# Autodesk Inventor assembly: DelrinX-Wheel-Top_MIR
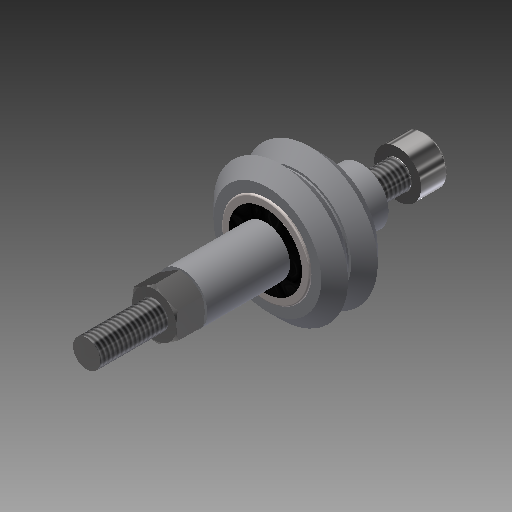
[picture p0: Inventor's stored thumbnail of the model, 512x512]
Saved by Autodesk Inventor 2017 (Build 210142000, 142)
## iProperties
Created: 2016-07-20
Part Number: DelrinX-Wheel-Top_MIR
Document SubType Name: Assembly
Designer: User
Author: User
## Documents named in this file (6)
- C:\All INVENTOR\SL-Inventor\SL-Beast 3D Printer\DelrinX-Wheel-Top_MIR.iam
- C:\All INVENTOR\SL-Inventor\SL-Beast 3D Printer\DelrinWheel_MIR.iam
- C:\All INVENTOR\SL-Inventor\SL-Beast 3D Printer\Long-Spacer_MIR.ipt
- C:\All INVENTOR\SL-Inventor\SL-Beast 3D Printer\ANSI B18.3.1M - M5x0.8 x 60NEW_MIR.ipt
- C:\All INVENTOR\SL-Inventor\SL-Beast 3D Printer\en-US\ANSI B 18.2.4.1 M(1)\ANSI B 18.2.4.1 M - M5 x 0.8Style 2.ipt
- C:\All INVENTOR\SL-Inventor\SL-Beast 3D Printer\Small-Aluminium-Spacer_MIR1.ipt
## Components (5 placed, 5 different names)
1. DelrinWheel_MIR:1 [sub-assembly] — Mate:2, Mate:1, Flush:1
2. Long-Spacer_MIR:1 — Insert:1
3. ANSI B18.3.1M - M5x0.8 x 60NEW_MIR:1 — Mate:2, Mate:1
4. Hex Nut Metric M5 x 0.8:1 — Insert:1
5. Small-Aluminium-Spacer_MIR1:1 — Flush:1
## Relationships (4: Mate 3, Insert 1)
- Mate:2 (13 mm): DelrinWheel_MIR:1 ↔ ANSI B18.3.1M - M5x0.8 x 60NEW_MIR:1
- Mate:1: DelrinWheel_MIR:1 ↔ ANSI B18.3.1M - M5x0.8 x 60NEW_MIR:1
- Insert:1: Long-Spacer_MIR:1 ↔ Hex Nut Metric M5 x 0.8:1
- Flush:1 [Mate]: DelrinWheel_MIR:1 ↔ Small-Aluminium-Spacer_MIR1:1
